# Autodesk Inventor assembly: PLANTA
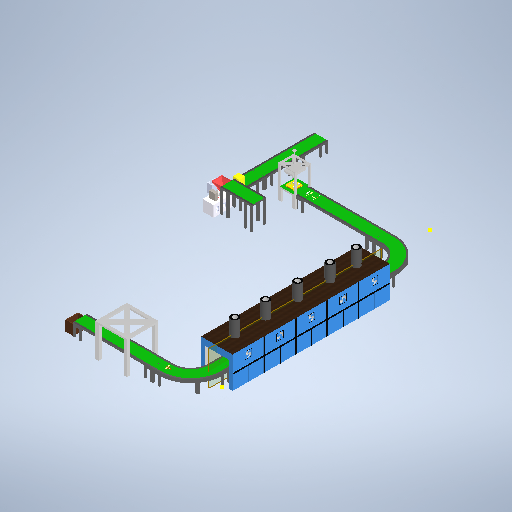
[picture p0: Inventor's stored thumbnail of the model, 512x512]
Saved by Autodesk Inventor 2025.2 (Build 292293000, 293)
## iProperties
Created: 2025-02-15
Part Number: PLANTA
Document SubType Name: Assembly
Designer: hmont
Author: hmont
## Documents named in this file (14)
- C:\Users\hmont\OneDrive\Desktop\2024-2\Automatizacion de Procesos de Manufactura\Modelado\PLANTA FINAL\PLANTA.iam
- C:\Users\hmont\OneDrive\Desktop\2024-2\Automatizacion de Procesos de Manufactura\Modelado\Mezcladora_Enfriadora\extrusora.iam
- C:\Users\hmont\OneDrive\Desktop\2024-2\Automatizacion de Procesos de Manufactura\Modelado\Bandas\Banda_R_2m_700.ipt
- C:\Users\hmont\OneDrive\Desktop\2024-2\Automatizacion de Procesos de Manufactura\Modelado\Bandas\Banda_R_2m_1500.ipt
- C:\Users\hmont\OneDrive\Desktop\2024-2\Automatizacion de Procesos de Manufactura\Modelado\Bandas\Banda_R_5m.ipt
- C:\Users\hmont\OneDrive\Desktop\2024-2\Automatizacion de Procesos de Manufactura\Modelado\Bandas\Rodillo_C_2,5m.ipt
- C:\Users\hmont\OneDrive\Desktop\2024-2\Automatizacion de Procesos de Manufactura\Modelado\Cortadora\Estacion_Corte.iam
- C:\Users\hmont\OneDrive\Desktop\2024-2\Automatizacion de Procesos de Manufactura\Modelado\Enfriadora\Enfriamiento_Transporte.ipt
- C:\Users\hmont\OneDrive\Desktop\2024-2\Automatizacion de Procesos de Manufactura\Modelado\Inspeccion de Calidad\Inspeccion_Calidad.iam
- C:\Users\hmont\OneDrive\Desktop\2024-2\Automatizacion de Procesos de Manufactura\Modelado\Camion\Caja.ipt
- C:\Users\hmont\OneDrive\Desktop\2024-2\Automatizacion de Procesos de Manufactura\Modelado\Procesos\Lamina.ipt
- C:\Users\hmont\OneDrive\Desktop\2024-2\Automatizacion de Procesos de Manufactura\Modelado\Procesos\Material.ipt
- C:\Users\hmont\Downloads\wooden-toy-plane-biplane-pdf-1.snapshot.3\ToyPlaneAssembly\ToyPlaneAssembly\ToyPlaneAssembly.iam
- C:\Users\hmont\OneDrive\Desktop\2024-2\Automatizacion de Procesos de Manufactura\Juguete\Placa_Juguete\Placa_Juguete\Placa_Juguete.ipt
## Components (19 placed, 13 different names)
1. extrusora:1 [sub-assembly]
2. Banda_R_2m_700:1 — Rígido:2
3. Banda_R_2m_1500:1
4. Banda_R_5m:1 — Rígido:1, Rígido:10
5. Rodillo_C_2,5m:1 — Rígido:1, Rígido:9
6. Banda_R_2m_700:2 — Rígido:2, Rígido:8
7. Banda_R_5m:2 — Rígido:5, Rígido:9
8. Enfriamiento_Transporte:1
9. Banda_R_5m:3 — Rígido:5, Rígido:6
10. Rodillo_C_2,5m:2 — Rígido:6, Rígido:7
11. Inspeccion_Calidad:1 [sub-assembly]
12. Banda_R_5m:4 — Rígido:7
13. Banda_R_2m_700:3 — Rígido:8
14. Estacion_Corte:1 [sub-assembly] — Rígido:10
15. Caja:1
16. Lamina:1
17. Material:1
18. ToyPlaneAssembly:1 [sub-assembly]
19. Placa_Juguete:1
## Relationships (8: WeldJoint 8)
- Rígido:1 [WeldJoint]: Banda_R_5m:1 ↔ Rodillo_C_2,5m:1
- Rígido:2 [WeldJoint]: Banda_R_2m_700:1 ↔ Banda_R_2m_700:2
- Rígido:5 [WeldJoint]: Banda_R_5m:2 ↔ Banda_R_5m:3
- Rígido:6 [WeldJoint]: Banda_R_5m:3 ↔ Rodillo_C_2,5m:2
- Rígido:7 [WeldJoint]: Rodillo_C_2,5m:2 ↔ Banda_R_5m:4
- Rígido:8 [WeldJoint]: Banda_R_2m_700:2 ↔ Banda_R_2m_700:3
- Rígido:9 [WeldJoint]: Rodillo_C_2,5m:1 ↔ Banda_R_5m:2
- Rígido:10 [WeldJoint]: Banda_R_5m:1 ↔ Estacion_Corte:1
